# Autodesk Inventor assembly: FRAME
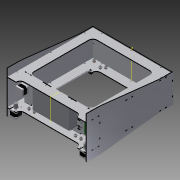
[picture p0: Inventor's stored thumbnail of the model, 180x180]
Saved by Autodesk Inventor 2013 (Build 170138000, 138)
## iProperties
Created: 2014-06-21
Part Number: FRAME
Document SubType Name: Assembly
Designer: employee
Author: employee
## Documents named in this file (27)
- C:\Users\employee\Desktop\ConceptFORGE\ConceptFORGE\CoreXZ\FRAME.iam
- C:\Users\employee\Desktop\ConceptFORGE\ConceptFORGE\CoreXZ\BACK PLATE.ipt
- C:\Users\employee\Desktop\ConceptFORGE\ConceptFORGE\CoreXZ\M8X290 ROD.ipt
- C:\Users\employee\Desktop\ConceptFORGE\ConceptFORGE\CoreXZ\RETAINER.ipt
- C:\Users\employee\Desktop\ConceptFORGE\ConceptFORGE\CoreXZ\ZIP TIE GANTRY ROD.ipt
- C:\Users\employee\Desktop\ConceptFORGE\ConceptFORGE\CoreXZ\M3 SQUARE NUT.ipt
- C:\Users\employee\Desktop\ConceptFORGE\ConceptFORGE\CoreXZ\FRONT PLATE.ipt
- C:\Users\employee\Desktop\ConceptFORGE\ConceptFORGE\CoreXZ\TOP PLATE.ipt
- C:\Users\employee\Desktop\ConceptFORGE\ConceptFORGE\CoreXZ\M3X12.ipt
- C:\Users\employee\Desktop\ConceptFORGE\ConceptFORGE\CoreXZ\SIDE PLATE.ipt
- C:\Users\employee\Desktop\ConceptFORGE\ConceptFORGE\CoreXZ\BOTTOM PLATE.ipt
- C:\Users\employee\Desktop\ConceptFORGE\ConceptFORGE\CoreXZ\LM8UU.ipt
- C:\Users\employee\Desktop\ConceptFORGE\ConceptFORGE\CoreXZ\ZIP TIE Y BEARINGS.ipt
- C:\Users\employee\Desktop\ConceptFORGE\ConceptFORGE\CoreXZ\STEPPER.ipt
- C:\Users\employee\Desktop\ConceptFORGE\ConceptFORGE\CoreXZ\SPOOL.ipt
- C:\Users\employee\Desktop\ConceptFORGE\ConceptFORGE\CoreXZ\M3X10.ipt
- C:\Users\employee\Desktop\ConceptFORGE\ConceptFORGE\CoreXZ\PULLEY ASSEMBLY.iam
- C:\Users\employee\Desktop\ConceptFORGE\ConceptFORGE\CoreXZ\BED TENSIONER MOUNT.ipt
- C:\Users\employee\Desktop\ConceptFORGE\ConceptFORGE\CoreXZ\TUNING PEG.ipt
- C:\Users\employee\Desktop\ConceptFORGE\ConceptFORGE\CoreXZ\M2X10.ipt
- C:\Users\employee\Desktop\ConceptFORGE\ConceptFORGE\CoreXZ\TUNING PEG RETAINER.ipt
- C:\Users\employee\Desktop\ConceptFORGE\ConceptFORGE\CoreXZ\M5X20.ipt
- C:\Users\employee\Desktop\ConceptFORGE\ConceptFORGE\CoreXZ\M5 NUT.ipt
- C:\Users\employee\Desktop\ConceptFORGE\ConceptFORGE\CoreXZ\POWER SUPPLY.ipt
- C:\Users\employee\Desktop\ConceptFORGE\ConceptFORGE\CoreXZ\M4x12.ipt
- C:\Users\employee\Desktop\ConceptFORGE\ConceptFORGE\CoreXZ\STANDOFF.ipt
- C:\Users\employee\Desktop\ConceptFORGE\ConceptFORGE\CoreXZ\ELECTRONICS.ipt
## Components (137 placed, 26 different names)
1. BACK PLATE:1 — Mate:1, Mate:2, Tangent:1, Tangent:2, Tangent:3, Mate:3, Mate:4, Mate:5, Mate:6, Flush:1, Flush:2, Flush:3, Flush:4, Flush:5, Flush:6, Flush:7, Flush:8, Angle:1, Angle:2, Tangent:4, Angle:3, Angle:4, Mate:7, Mate:8, Flush:9, Mate:9, Mate:10, Mate:11, Mate:12, Mate:13, Mate:14, Mate:15, Mate:16, Mate:17, Mate:18, Mate:19, Mate:20, Mate:21, Mate:22, Mate:23, Mate:24, Flush:10, Flush:11, Flush:12, Flush:13, Flush:14, Flush:15, Flush:16, Flush:17, Flush:18, Flush:19, Flush:20, Mate:25, Flush:21, Mate:59, Mate:60, Mate:61, Mate:62, Flush:40, Flush:41, Insert:27, Insert:29, Insert:31, Insert:46, Insert:47, Angle:13, Angle:14, Angle:15, Insert:55, Insert:56, Insert:57, Insert:58, Insert:59, Insert:60, Insert:61, Insert:62, Insert:63, Insert:64, Insert:65, Insert:66, Insert:67, Insert:68, Insert:69, Insert:70, Insert:71, Insert:72
2. M8X290 ROD:1 — Mate:1, Tangent:2, Tangent:3, Insert:3, Insert:4
3. M8X290 ROD:2 — Mate:2, Tangent:1, Insert:1, Insert:2, Tangent:4
4. RETAINER:1 — Mate:3, Flush:4, Flush:7
5. RETAINER:2 — Mate:5, Flush:1, Flush:8
6. RETAINER:3 — Mate:4, Flush:3, Flush:5
7. RETAINER:4 — Mate:6, Flush:2, Flush:6
8. ZIP TIE GANTRY ROD:2 — Insert:1, Angle:3
9. ZIP TIE GANTRY ROD:3 — Insert:2, Angle:4
10. ZIP TIE GANTRY ROD:4 — Insert:3, Angle:1
11. ZIP TIE GANTRY ROD:5 — Insert:4, Angle:2
12. M3 SQUARE NUT:1 — Mate:7, Mate:8, Flush:9, Flush:16
13. M3 SQUARE NUT:2 — Mate:9, Mate:10, Flush:17
14. M3 SQUARE NUT:3 — Mate:11, Mate:12, Flush:18
15. M3 SQUARE NUT:4 — Mate:13, Mate:14, Flush:15
16. M3 SQUARE NUT:5 — Mate:15, Mate:16, Flush:14
17. M3 SQUARE NUT:6 — Mate:17, Mate:18, Flush:13
18. M3 SQUARE NUT:7 — Mate:19, Mate:20, Flush:12
19. M3 SQUARE NUT:8 — Mate:21, Mate:24, Flush:10
20. M3 SQUARE NUT:9 — Mate:22, Mate:23, Flush:11
21. FRONT PLATE:1 — Flush:19, Flush:20, Mate:25, Flush:22, Mate:30, Mate:31, Mate:32, Mate:33, Mate:34, Mate:35, Mate:36, Mate:37, Mate:38, Mate:39, Flush:25, Mate:40, Flush:26, Mate:41, Flush:27, Mate:42, Flush:28, Mate:43, Flush:29, Mate:44, Flush:30, Mate:45, Flush:31, Mate:46, Flush:32, Mate:47, Flush:33, Mate:48, Flush:36, Mate:53, Flush:37, Mate:55, Mate:56, Mate:57, Flush:38, Mate:58, Flush:39, Insert:32, Insert:34, Insert:36, Mate:81, Mate:84
22. TOP PLATE:1 — Flush:21, Insert:5, Insert:6, Insert:7, Insert:8, Insert:9, Insert:10, Mate:26, Mate:27, Flush:23, Mate:28, Mate:29, Flush:24
23. M3X12:1 — Insert:5
24. M3X12:2 — Insert:6
25. M3X12:3 — Insert:7
26. M3X12:4 — Insert:10
27. M3X12:5 — Insert:9
28. M3X12:6 — Insert:8
29. SIDE PLATE:1 — Flush:22, Flush:34, Flush:35, Insert:18, Insert:19, Insert:20, Insert:21, Insert:22, Insert:23, Insert:24, Mate:54, Insert:25, Angle:9, Angle:10, Angle:11, Angle:12, Mate:83
30. M3 SQUARE NUT:10 — Mate:28, Mate:29, Flush:24
31. M3 SQUARE NUT:11 — Mate:26, Mate:27, Flush:23
32. M3 SQUARE NUT:12 — Mate:38, Mate:39, Flush:25
33. M3 SQUARE NUT:13 — Mate:31, Mate:46, Flush:32
34. M3 SQUARE NUT:14 — Mate:30, Mate:47, Flush:33
35. M3 SQUARE NUT:15 — Mate:32, Mate:45, Flush:31
36. M3 SQUARE NUT:16 — Mate:33, Mate:44, Flush:30
37. M3 SQUARE NUT:17 — Mate:35, Mate:42, Flush:28
38. M3 SQUARE NUT:18 — Mate:34, Mate:43, Flush:29
39. M3 SQUARE NUT:19 — Mate:36, Mate:40, Flush:26
40. M3 SQUARE NUT:20 — Mate:37, Mate:41, Flush:27
41. SIDE PLATE:2 — Mate:48, Flush:34, Flush:35, Insert:11, Insert:12, Insert:13, Insert:14, Insert:15, Insert:16, Insert:17, Insert:26, Angle:5, Angle:6, Angle:7, Angle:8
42. M3X12:7 — Insert:11
43. M3X12:8 — Insert:12
44. M3X12:9 — Insert:13
45. M3X12:10 — Insert:14
46. M3X12:11 — Insert:15
47. M3X12:12 — Insert:16
48. M3X12:13 — Insert:17
49. M3X12:14 — Insert:18
50. M3X12:15 — Insert:19
51. M3X12:16 — Insert:20
52. M3X12:17 — Insert:21
53. M3X12:18 — Insert:22
54. M3X12:19 — Insert:23
55. M3X12:20 — Insert:24
56. BOTTOM PLATE:1 — Flush:36, Mate:49, Mate:50, Mate:51, Mate:52, Tangent:5, Tangent:6, Tangent:7, Tangent:8, Tangent:9, Tangent:11, Tangent:12, Tangent:13, Mate:53, Mate:54, Flush:37, Mate:63, Mate:64, Flush:42, Mate:65, Mate:66, Flush:43, Mate:67, Mate:68, Flush:44, Mate:69, Mate:70, Flush:45, Mate:71, Mate:72, Flush:46, Mate:73, Mate:74, Flush:47, Mate:75, Mate:76, Flush:48, Mate:77, Mate:78, Flush:49, Insert:28, Insert:30, Insert:33, Insert:35, Insert:45, Insert:51, Insert:52, Insert:53, Insert:54, Insert:73, Insert:74, Insert:75, Insert:76, Insert:82, Insert:83, Mate:79, Insert:84, Insert:85, Insert:86, Insert:87, Mate:82
57. LM8UU:1 — Mate:49, Tangent:9, Tangent:13, Insert:39, Insert:40
58. LM8UU:2 — Mate:50, Tangent:11, Tangent:12, Insert:37, Insert:38
59. LM8UU:3 — Mate:51, Tangent:7, Tangent:8, Insert:43, Insert:44
60. LM8UU:4 — Mate:52, Tangent:5, Tangent:6, Insert:41, Insert:42
61. M3 SQUARE NUT:21 — Mate:55, Mate:57, Flush:38
62. M3 SQUARE NUT:22 — Mate:56, Mate:58, Flush:39
63. M3 SQUARE NUT:23 — Mate:59, Mate:62, Flush:40
64. M3 SQUARE NUT:24 — Mate:60, Mate:61, Flush:41
65. M3 SQUARE NUT:25 — Mate:75, Mate:76, Flush:48
66. M3 SQUARE NUT:26 — Mate:73, Mate:74, Flush:47
67. M3 SQUARE NUT:27 — Mate:71, Mate:72, Flush:46
68. M3 SQUARE NUT:28 — Mate:63, Mate:64, Flush:42
69. M3 SQUARE NUT:29 — Mate:65, Mate:66, Flush:43
70. M3 SQUARE NUT:30 — Mate:67, Mate:68, Flush:44
71. M3 SQUARE NUT:31 — Mate:69, Mate:70, Flush:45
72. M3 SQUARE NUT:32 — Mate:77, Mate:78, Flush:49
73. M3X12:21 — Insert:25
74. M3X12:22 — Insert:26
75. M3X12:23 — Insert:27
76. M3X12:24 — Insert:28
77. M3X12:25 — Insert:29
78. M3X12:26 — Insert:30
79. M3X12:27 — Insert:31
80. M3X12:28 — Insert:32
81. M3X12:29 — Insert:33
82. M3X12:30 — Insert:34
83. M3X12:31 — Insert:35
84. M3X12:32 — Insert:36
85. ZIP TIE Y BEARINGS:1 — Insert:37, Angle:5
86. ZIP TIE Y BEARINGS:2 — Insert:38, Angle:7
87. ZIP TIE Y BEARINGS:3 — Insert:39, Angle:6
88. ZIP TIE Y BEARINGS:4 — Insert:40, Angle:8
89. ZIP TIE Y BEARINGS:5 — Insert:41, Angle:10
90. ZIP TIE Y BEARINGS:6 — Insert:42, Angle:12
91. ZIP TIE Y BEARINGS:7 — Insert:43, Angle:9
92. ZIP TIE Y BEARINGS:8 — Insert:44, Angle:11
93. STEPPER:1 — Insert:45, Angle:15, Insert:48
94. STEPPER:2 — Insert:46, Angle:14, Insert:49
95. STEPPER:3 — Insert:47, Angle:13, Insert:50
96. SPOOL:1 — Insert:48
97. SPOOL:2 — Insert:50
98. SPOOL:3 — Insert:49
99. M3X10:1 — Insert:60
100. M3X10:2 — Insert:59
101. M3X10:3 — Insert:61
102. M3X10:4 — Insert:62
103. M3X10:5 — Insert:58
104. M3X10:6 — Insert:57
105. M3X10:7 — Insert:56
106. M3X10:8 — Insert:55
107. M3X10:9 — Insert:54
108. M3X10:10 — Insert:53
109. M3X10:11 — Insert:51
110. M3X10:12 — Insert:52
111. PULLEY ASSEMBLY:1 [sub-assembly] — Insert:63
112. PULLEY ASSEMBLY:2 [sub-assembly] — Insert:64
113. PULLEY ASSEMBLY:3 [sub-assembly] — Insert:65
114. PULLEY ASSEMBLY:4 [sub-assembly] — Insert:66
115. PULLEY ASSEMBLY:5 [sub-assembly] — Insert:69
116. PULLEY ASSEMBLY:6 [sub-assembly] — Insert:70
117. PULLEY ASSEMBLY:7 [sub-assembly] — Insert:68
118. PULLEY ASSEMBLY:8 [sub-assembly] — Insert:72
119. PULLEY ASSEMBLY:9 [sub-assembly] — Insert:71
120. PULLEY ASSEMBLY:10 [sub-assembly] — Insert:67
121. PULLEY ASSEMBLY:11 [sub-assembly] — Insert:73
122. PULLEY ASSEMBLY:12 [sub-assembly] — Insert:74
123. BED TENSIONER MOUNT:1 — Insert:75, Insert:76, Insert:77, Angle:16, Insert:79, Insert:80, Insert:81
124. TUNING PEG:1 — Insert:77, Angle:16, Insert:78
125. M2X10:1 — Insert:78
126. TUNING PEG RETAINER:1 — Insert:79
127. M5X20:1 — Insert:80
128. M5X20:2 — Insert:81
129. M5 NUT:1 — Insert:82
130. M5 NUT:2 — Insert:83
131. POWER SUPPLY:1 — Mate:79, Mate:80, Mate:81
132. Forged Socket Head Cap Screw - Metric M4x0.7 x 12:1 — Insert:84
133. Forged Socket Head Cap Screw - Metric M4x0.7 x 12:2 — Insert:85
134. Forged Socket Head Cap Screw - Metric M4x0.7 x 12:3 — Insert:86
135. Forged Socket Head Cap Screw - Metric M4x0.7 x 12:4 — Insert:87
136. STANDOFF:1 — Mate:82, Insert:88, Insert:89
137. ELECTRONICS:1 — Insert:88, Insert:89, Mate:83, Mate:84
## Relationships (250: Insert 89, Mate 84, Flush 49, Angle 16, Tangent 12)
- Mate:1: BACK PLATE:1 ↔ M8X290 ROD:1
- Mate:2: BACK PLATE:1 ↔ M8X290 ROD:2
- Tangent:1: BACK PLATE:1 ↔ M8X290 ROD:2
- Tangent:2: BACK PLATE:1 ↔ M8X290 ROD:1
- Tangent:3: BACK PLATE:1 ↔ M8X290 ROD:1
- Mate:3: BACK PLATE:1 ↔ RETAINER:1
- Mate:4: BACK PLATE:1 ↔ RETAINER:3
- Mate:5: BACK PLATE:1 ↔ RETAINER:2
- Mate:6: BACK PLATE:1 ↔ RETAINER:4
- Flush:1: BACK PLATE:1 ↔ RETAINER:2
- Flush:2: BACK PLATE:1 ↔ RETAINER:4
- Flush:3: BACK PLATE:1 ↔ RETAINER:3
- Flush:4: BACK PLATE:1 ↔ RETAINER:1
- Flush:5: BACK PLATE:1 ↔ RETAINER:3
- Flush:6: BACK PLATE:1 ↔ RETAINER:4
- Flush:7: BACK PLATE:1 ↔ RETAINER:1
- Flush:8: BACK PLATE:1 ↔ RETAINER:2
- Insert:1 (3.25 mm): M8X290 ROD:2 ↔ ZIP TIE GANTRY ROD:2
- Insert:2 (3.25 mm): M8X290 ROD:2 ↔ ZIP TIE GANTRY ROD:3
- Insert:3 (3.25 mm): M8X290 ROD:1 ↔ ZIP TIE GANTRY ROD:4
- Insert:4 (3.25 mm): M8X290 ROD:1 ↔ ZIP TIE GANTRY ROD:5
- Angle:1 (0 deg): BACK PLATE:1 ↔ ZIP TIE GANTRY ROD:4
- Angle:2 (0 deg): BACK PLATE:1 ↔ ZIP TIE GANTRY ROD:5
- Tangent:4: BACK PLATE:1 ↔ M8X290 ROD:2
- Angle:3 (0 deg): BACK PLATE:1 ↔ ZIP TIE GANTRY ROD:2
- Angle:4 (0 deg): BACK PLATE:1 ↔ ZIP TIE GANTRY ROD:3
- Mate:7: BACK PLATE:1 ↔ M3 SQUARE NUT:1
- Mate:8: BACK PLATE:1 ↔ M3 SQUARE NUT:1
- Flush:9: BACK PLATE:1 ↔ M3 SQUARE NUT:1
- Mate:9: BACK PLATE:1 ↔ M3 SQUARE NUT:2
- Mate:10: BACK PLATE:1 ↔ M3 SQUARE NUT:2
- Mate:11: BACK PLATE:1 ↔ M3 SQUARE NUT:3
- Mate:12: BACK PLATE:1 ↔ M3 SQUARE NUT:3
- Mate:13: BACK PLATE:1 ↔ M3 SQUARE NUT:4
- Mate:14: BACK PLATE:1 ↔ M3 SQUARE NUT:4
- Mate:15: BACK PLATE:1 ↔ M3 SQUARE NUT:5
- Mate:16: BACK PLATE:1 ↔ M3 SQUARE NUT:5
- Mate:17: BACK PLATE:1 ↔ M3 SQUARE NUT:6
- Mate:18: BACK PLATE:1 ↔ M3 SQUARE NUT:6
- Mate:19: BACK PLATE:1 ↔ M3 SQUARE NUT:7
- Mate:20: BACK PLATE:1 ↔ M3 SQUARE NUT:7
- Mate:21: BACK PLATE:1 ↔ M3 SQUARE NUT:8
- Mate:22: BACK PLATE:1 ↔ M3 SQUARE NUT:9
- Mate:23: BACK PLATE:1 ↔ M3 SQUARE NUT:9
- Mate:24: BACK PLATE:1 ↔ M3 SQUARE NUT:8
- Flush:10: BACK PLATE:1 ↔ M3 SQUARE NUT:8
- Flush:11: BACK PLATE:1 ↔ M3 SQUARE NUT:9
- Flush:12: BACK PLATE:1 ↔ M3 SQUARE NUT:7
- Flush:13: BACK PLATE:1 ↔ M3 SQUARE NUT:6
- Flush:14: BACK PLATE:1 ↔ M3 SQUARE NUT:5
- Flush:15: BACK PLATE:1 ↔ M3 SQUARE NUT:4
- Flush:16: BACK PLATE:1 ↔ M3 SQUARE NUT:1
- Flush:17: BACK PLATE:1 ↔ M3 SQUARE NUT:2
- Flush:18: BACK PLATE:1 ↔ M3 SQUARE NUT:3
- Flush:19: BACK PLATE:1 ↔ FRONT PLATE:1
- Flush:20: BACK PLATE:1 ↔ FRONT PLATE:1
- Mate:25 (150 mm): BACK PLATE:1 ↔ FRONT PLATE:1
- Flush:21: BACK PLATE:1 ↔ TOP PLATE:1
- Insert:5: TOP PLATE:1 ↔ M3X12:1
- Insert:6: TOP PLATE:1 ↔ M3X12:2
- Insert:7: TOP PLATE:1 ↔ M3X12:3
- Insert:8: TOP PLATE:1 ↔ M3X12:6
- Insert:9: TOP PLATE:1 ↔ M3X12:5
- Insert:10: TOP PLATE:1 ↔ M3X12:4
- Flush:22: FRONT PLATE:1 ↔ SIDE PLATE:1
- Mate:26: TOP PLATE:1 ↔ M3 SQUARE NUT:11
- Mate:27: TOP PLATE:1 ↔ M3 SQUARE NUT:11
- Flush:23: TOP PLATE:1 ↔ M3 SQUARE NUT:11
- Mate:28: TOP PLATE:1 ↔ M3 SQUARE NUT:10
- Mate:29: TOP PLATE:1 ↔ M3 SQUARE NUT:10
- Flush:24: TOP PLATE:1 ↔ M3 SQUARE NUT:10
- Mate:30: FRONT PLATE:1 ↔ M3 SQUARE NUT:14
- Mate:31: FRONT PLATE:1 ↔ M3 SQUARE NUT:13
- Mate:32: FRONT PLATE:1 ↔ M3 SQUARE NUT:15
- Mate:33: FRONT PLATE:1 ↔ M3 SQUARE NUT:16
- Mate:34: FRONT PLATE:1 ↔ M3 SQUARE NUT:18
- Mate:35: FRONT PLATE:1 ↔ M3 SQUARE NUT:17
- Mate:36: FRONT PLATE:1 ↔ M3 SQUARE NUT:19
- Mate:37: FRONT PLATE:1 ↔ M3 SQUARE NUT:20
- Mate:38: FRONT PLATE:1 ↔ M3 SQUARE NUT:12
- Mate:39: FRONT PLATE:1 ↔ M3 SQUARE NUT:12
- Flush:25: FRONT PLATE:1 ↔ M3 SQUARE NUT:12
- Mate:40: FRONT PLATE:1 ↔ M3 SQUARE NUT:19
- Flush:26: FRONT PLATE:1 ↔ M3 SQUARE NUT:19
- Mate:41: FRONT PLATE:1 ↔ M3 SQUARE NUT:20
- Flush:27: FRONT PLATE:1 ↔ M3 SQUARE NUT:20
- Mate:42: FRONT PLATE:1 ↔ M3 SQUARE NUT:17
- Flush:28: FRONT PLATE:1 ↔ M3 SQUARE NUT:17
- Mate:43: FRONT PLATE:1 ↔ M3 SQUARE NUT:18
- Flush:29: FRONT PLATE:1 ↔ M3 SQUARE NUT:18
- Mate:44: FRONT PLATE:1 ↔ M3 SQUARE NUT:16
- Flush:30: FRONT PLATE:1 ↔ M3 SQUARE NUT:16
- Mate:45: FRONT PLATE:1 ↔ M3 SQUARE NUT:15
- Flush:31: FRONT PLATE:1 ↔ M3 SQUARE NUT:15
- Mate:46: FRONT PLATE:1 ↔ M3 SQUARE NUT:13
- Flush:32: FRONT PLATE:1 ↔ M3 SQUARE NUT:13
- Mate:47: FRONT PLATE:1 ↔ M3 SQUARE NUT:14
- Flush:33: FRONT PLATE:1 ↔ M3 SQUARE NUT:14
- Mate:48: FRONT PLATE:1 ↔ SIDE PLATE:2
- Flush:34: SIDE PLATE:1 ↔ SIDE PLATE:2
- Flush:35: SIDE PLATE:1 ↔ SIDE PLATE:2
- Insert:11: SIDE PLATE:2 ↔ M3X12:7
- Insert:12: SIDE PLATE:2 ↔ M3X12:8
- Insert:13: SIDE PLATE:2 ↔ M3X12:9
- Insert:14: SIDE PLATE:2 ↔ M3X12:10
- Insert:15: SIDE PLATE:2 ↔ M3X12:11
- Insert:16: SIDE PLATE:2 ↔ M3X12:12
- Insert:17: SIDE PLATE:2 ↔ M3X12:13
- Insert:18: SIDE PLATE:1 ↔ M3X12:14
- Insert:19: SIDE PLATE:1 ↔ M3X12:15
- Insert:20: SIDE PLATE:1 ↔ M3X12:16
- Insert:21: SIDE PLATE:1 ↔ M3X12:17
- Insert:22: SIDE PLATE:1 ↔ M3X12:18
- Insert:23: SIDE PLATE:1 ↔ M3X12:19
- Insert:24: SIDE PLATE:1 ↔ M3X12:20
- Flush:36: FRONT PLATE:1 ↔ BOTTOM PLATE:1
- Mate:49: BOTTOM PLATE:1 ↔ LM8UU:1
- Mate:50: BOTTOM PLATE:1 ↔ LM8UU:2
- Mate:51: BOTTOM PLATE:1 ↔ LM8UU:3
- Mate:52: BOTTOM PLATE:1 ↔ LM8UU:4
- Tangent:5: BOTTOM PLATE:1 ↔ LM8UU:4
- Tangent:6: BOTTOM PLATE:1 ↔ LM8UU:4
- Tangent:7: BOTTOM PLATE:1 ↔ LM8UU:3
- Tangent:8: BOTTOM PLATE:1 ↔ LM8UU:3
- Tangent:9: BOTTOM PLATE:1 ↔ LM8UU:1
- Tangent:11: BOTTOM PLATE:1 ↔ LM8UU:2
- Tangent:12: BOTTOM PLATE:1 ↔ LM8UU:2
- Tangent:13: BOTTOM PLATE:1 ↔ LM8UU:1
- Mate:53: FRONT PLATE:1 ↔ BOTTOM PLATE:1
- Mate:54: SIDE PLATE:1 ↔ BOTTOM PLATE:1
- Flush:37: FRONT PLATE:1 ↔ BOTTOM PLATE:1
- Mate:55: FRONT PLATE:1 ↔ M3 SQUARE NUT:21
- Mate:56: FRONT PLATE:1 ↔ M3 SQUARE NUT:22
- Mate:57: FRONT PLATE:1 ↔ M3 SQUARE NUT:21
- Flush:38: FRONT PLATE:1 ↔ M3 SQUARE NUT:21
- Mate:58: FRONT PLATE:1 ↔ M3 SQUARE NUT:22
- Flush:39: FRONT PLATE:1 ↔ M3 SQUARE NUT:22
- Mate:59: BACK PLATE:1 ↔ M3 SQUARE NUT:23
- Mate:60: BACK PLATE:1 ↔ M3 SQUARE NUT:24
- Mate:61: BACK PLATE:1 ↔ M3 SQUARE NUT:24
- Mate:62: BACK PLATE:1 ↔ M3 SQUARE NUT:23
- Flush:40: BACK PLATE:1 ↔ M3 SQUARE NUT:23
- Flush:41: BACK PLATE:1 ↔ M3 SQUARE NUT:24
- Mate:63: BOTTOM PLATE:1 ↔ M3 SQUARE NUT:28
- Mate:64: BOTTOM PLATE:1 ↔ M3 SQUARE NUT:28
- Flush:42: BOTTOM PLATE:1 ↔ M3 SQUARE NUT:28
- Mate:65: BOTTOM PLATE:1 ↔ M3 SQUARE NUT:29
- Mate:66: BOTTOM PLATE:1 ↔ M3 SQUARE NUT:29
- Flush:43: BOTTOM PLATE:1 ↔ M3 SQUARE NUT:29
- Mate:67: BOTTOM PLATE:1 ↔ M3 SQUARE NUT:30
- Mate:68: BOTTOM PLATE:1 ↔ M3 SQUARE NUT:30
- Flush:44: BOTTOM PLATE:1 ↔ M3 SQUARE NUT:30
- Mate:69: BOTTOM PLATE:1 ↔ M3 SQUARE NUT:31
- Mate:70: BOTTOM PLATE:1 ↔ M3 SQUARE NUT:31
- Flush:45: BOTTOM PLATE:1 ↔ M3 SQUARE NUT:31
- Mate:71: BOTTOM PLATE:1 ↔ M3 SQUARE NUT:27
- Mate:72: BOTTOM PLATE:1 ↔ M3 SQUARE NUT:27
- Flush:46: BOTTOM PLATE:1 ↔ M3 SQUARE NUT:27
- Mate:73: BOTTOM PLATE:1 ↔ M3 SQUARE NUT:26
- Mate:74: BOTTOM PLATE:1 ↔ M3 SQUARE NUT:26
- Flush:47: BOTTOM PLATE:1 ↔ M3 SQUARE NUT:26
- Mate:75: BOTTOM PLATE:1 ↔ M3 SQUARE NUT:25
- Mate:76: BOTTOM PLATE:1 ↔ M3 SQUARE NUT:25
- Flush:48: BOTTOM PLATE:1 ↔ M3 SQUARE NUT:25
- Mate:77: BOTTOM PLATE:1 ↔ M3 SQUARE NUT:32
- Mate:78: BOTTOM PLATE:1 ↔ M3 SQUARE NUT:32
- Flush:49: BOTTOM PLATE:1 ↔ M3 SQUARE NUT:32
- Insert:25: SIDE PLATE:1 ↔ M3X12:21
- Insert:26: SIDE PLATE:2 ↔ M3X12:22
- Insert:27: BACK PLATE:1 ↔ M3X12:23
- Insert:28: BOTTOM PLATE:1 ↔ M3X12:24
- Insert:29: BACK PLATE:1 ↔ M3X12:25
- Insert:30: BOTTOM PLATE:1 ↔ M3X12:26
- Insert:31: BACK PLATE:1 ↔ M3X12:27
- Insert:32: FRONT PLATE:1 ↔ M3X12:28
- Insert:33: BOTTOM PLATE:1 ↔ M3X12:29
- Insert:34: FRONT PLATE:1 ↔ M3X12:30
- Insert:35: BOTTOM PLATE:1 ↔ M3X12:31
- Insert:36: FRONT PLATE:1 ↔ M3X12:32
- Insert:37 (3.25 mm): LM8UU:2 ↔ ZIP TIE Y BEARINGS:1
- Insert:38 (3.25 mm): LM8UU:2 ↔ ZIP TIE Y BEARINGS:2
- Insert:39 (3.25 mm): LM8UU:1 ↔ ZIP TIE Y BEARINGS:3
- Insert:40 (3.25 mm): LM8UU:1 ↔ ZIP TIE Y BEARINGS:4
- Angle:5 (0 deg): SIDE PLATE:2 ↔ ZIP TIE Y BEARINGS:1
- Angle:6 (0 deg): SIDE PLATE:2 ↔ ZIP TIE Y BEARINGS:3
- Angle:7 (0 deg): SIDE PLATE:2 ↔ ZIP TIE Y BEARINGS:2
- Angle:8 (0 deg): SIDE PLATE:2 ↔ ZIP TIE Y BEARINGS:4
- Insert:41 (3.25 mm): LM8UU:4 ↔ ZIP TIE Y BEARINGS:5
- Insert:42 (3.25 mm): LM8UU:4 ↔ ZIP TIE Y BEARINGS:6
- Insert:43 (3.25 mm): LM8UU:3 ↔ ZIP TIE Y BEARINGS:7
- Insert:44 (3.25 mm): LM8UU:3 ↔ ZIP TIE Y BEARINGS:8
- Angle:9 (0 deg): SIDE PLATE:1 ↔ ZIP TIE Y BEARINGS:7
- Angle:10 (0 deg): SIDE PLATE:1 ↔ ZIP TIE Y BEARINGS:5
- Angle:11 (0 deg): SIDE PLATE:1 ↔ ZIP TIE Y BEARINGS:8
- Angle:12 (0 deg): SIDE PLATE:1 ↔ ZIP TIE Y BEARINGS:6
- Insert:45: BOTTOM PLATE:1 ↔ STEPPER:1
- Insert:46: BACK PLATE:1 ↔ STEPPER:2
- Insert:47: BACK PLATE:1 ↔ STEPPER:3
- Angle:13 (0 deg): BACK PLATE:1 ↔ STEPPER:3
- Angle:14 (0 deg): BACK PLATE:1 ↔ STEPPER:2
- Angle:15 (0 deg): BACK PLATE:1 ↔ STEPPER:1
- Insert:48: STEPPER:1 ↔ SPOOL:1
- Insert:49: STEPPER:2 ↔ SPOOL:3
- Insert:50: STEPPER:3 ↔ SPOOL:2
- Insert:51: BOTTOM PLATE:1 ↔ M3X10:11
- Insert:52: BOTTOM PLATE:1 ↔ M3X10:12
- Insert:53: BOTTOM PLATE:1 ↔ M3X10:10
- Insert:54: BOTTOM PLATE:1 ↔ M3X10:9
- Insert:55: BACK PLATE:1 ↔ M3X10:8
- Insert:56: BACK PLATE:1 ↔ M3X10:7
- Insert:57: BACK PLATE:1 ↔ M3X10:6
- Insert:58: BACK PLATE:1 ↔ M3X10:5
- Insert:59: BACK PLATE:1 ↔ M3X10:2
- Insert:60: BACK PLATE:1 ↔ M3X10:1
- Insert:61: BACK PLATE:1 ↔ M3X10:3
- Insert:62: BACK PLATE:1 ↔ M3X10:4
- Insert:63: BACK PLATE:1 ↔ PULLEY ASSEMBLY:1
- Insert:64: BACK PLATE:1 ↔ PULLEY ASSEMBLY:2
- Insert:65: BACK PLATE:1 ↔ PULLEY ASSEMBLY:3
- Insert:66: BACK PLATE:1 ↔ PULLEY ASSEMBLY:4
- Insert:67: BACK PLATE:1 ↔ PULLEY ASSEMBLY:10
- Insert:68: BACK PLATE:1 ↔ PULLEY ASSEMBLY:7
- Insert:69: BACK PLATE:1 ↔ PULLEY ASSEMBLY:5
- Insert:70: BACK PLATE:1 ↔ PULLEY ASSEMBLY:6
- Insert:71: BACK PLATE:1 ↔ PULLEY ASSEMBLY:9
- Insert:72: BACK PLATE:1 ↔ PULLEY ASSEMBLY:8
- Insert:73: BOTTOM PLATE:1 ↔ PULLEY ASSEMBLY:11
- Insert:74: BOTTOM PLATE:1 ↔ PULLEY ASSEMBLY:12
- Insert:75: BOTTOM PLATE:1 ↔ BED TENSIONER MOUNT:1
- Insert:76: BOTTOM PLATE:1 ↔ BED TENSIONER MOUNT:1
- Insert:77: BED TENSIONER MOUNT:1 ↔ TUNING PEG:1
- Angle:16 (0 deg): BED TENSIONER MOUNT:1 ↔ TUNING PEG:1
- Insert:78: TUNING PEG:1 ↔ M2X10:1
- Insert:79: BED TENSIONER MOUNT:1 ↔ TUNING PEG RETAINER:1
- Insert:80: BED TENSIONER MOUNT:1 ↔ M5X20:1
- Insert:81: BED TENSIONER MOUNT:1 ↔ M5X20:2
- Insert:82: BOTTOM PLATE:1 ↔ M5 NUT:1
- Insert:83: BOTTOM PLATE:1 ↔ M5 NUT:2
- Mate:79: BOTTOM PLATE:1 ↔ POWER SUPPLY:1
- Mate:80: POWER SUPPLY:1
- Mate:81: FRONT PLATE:1 ↔ POWER SUPPLY:1
- Insert:84: BOTTOM PLATE:1 ↔ Forged Socket Head Cap Screw - Metric M4x0.7 x 12:1
- Insert:85: BOTTOM PLATE:1 ↔ Forged Socket Head Cap Screw - Metric M4x0.7 x 12:2
- Insert:86: BOTTOM PLATE:1 ↔ Forged Socket Head Cap Screw - Metric M4x0.7 x 12:3
- Insert:87: BOTTOM PLATE:1 ↔ Forged Socket Head Cap Screw - Metric M4x0.7 x 12:4
- Mate:82: BOTTOM PLATE:1 ↔ STANDOFF:1
- Insert:88: STANDOFF:1 ↔ ELECTRONICS:1
- Insert:89: STANDOFF:1 ↔ ELECTRONICS:1
- Mate:83 (2 mm): SIDE PLATE:1 ↔ ELECTRONICS:1
- Mate:84 (2 mm): FRONT PLATE:1 ↔ ELECTRONICS:1
